# Autodesk Inventor assembly: PCB_board_box_reassemb
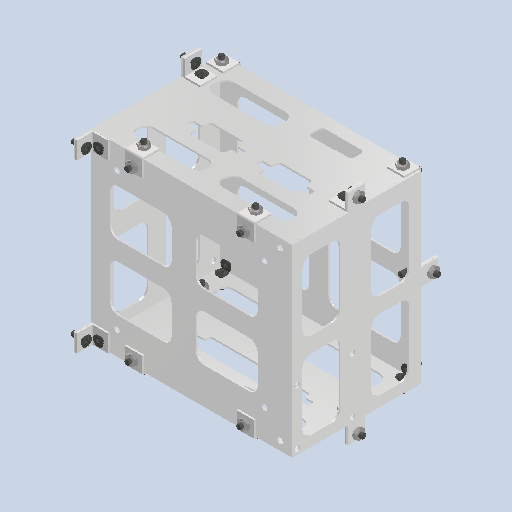
[picture p0: Inventor's stored thumbnail of the model, 512x512]
Saved by Autodesk Inventor 2023 (Build 270158000, 158)
## iProperties
Created: 2023-10-19
Part Number: PCB_board_box_reassemb
Document SubType Name: Assembly
Designer: 310611102
Author: 310611102
## Documents named in this file (10)
- C:\Users\310611102\Documents\Inventor\SSR\avionics_2023ver\electronics\shield box\shieldbox_ver2\PCB_board_box_reassemb.iam
- C:\Users\310611102\Documents\Inventor\SSR\avionics_2023ver\electronics\shield box\shieldbox_ver2\PCB_board_box_buttom.ipt
- C:\Users\310611102\Documents\Inventor\SSR\avionics_2023ver\electronics\shield box\shieldbox_ver2\PCB_board_box_front.ipt
- C:\Users\310611102\Documents\Inventor\SSR\avionics_2023ver\electronics\shield box\shieldbox_ver2\PCB_board_box_back.ipt
- C:\Users\310611102\Documents\Inventor\SSR\avionics_2023ver\electronics\shield box\shieldbox_ver2\PCB_board_box_right.ipt
- C:\Users\310611102\Documents\Inventor\SSR\avionics_2023ver\electronics\shield box\shieldbox_ver2\PCB_board_box_top.ipt
- C:\Users\310611102\Documents\Inventor\SSR\avionics_2023ver\electronics\shield box\shieldbox_ver2\PCB_board_box_left.ipt
- C:\Users\310611102\Documents\Inventor\SSR\avionics_2023ver\electronics\shield box\shieldbox_ver2\connector.ipt
- C:\Users\310611102\Documents\Inventor\SSR\avionics_2023ver\electronics\ISO 4032 - M3 - ISO.ipt
- C:\Users\310611102\Documents\Inventor\SSR\avionics_2023ver\electronics\ISO 10642 - M3 x  8.ipt
## Components (76 placed, 9 different names)
1. PCB_board_box_buttom:1 — Insert:16, Insert:18, Cylindrical:1, Cylindrical:3, Cylindrical:5, Cylindrical:9, Insert:53, Insert:55, Insert:57, Insert:59, Insert:85, Insert:87
2. PCB_board_box_front:1 — Insert:8, Insert:19, Cylindrical:4, Cylindrical:10, Cylindrical:13, Cylindrical:19, Insert:48, Insert:58, Insert:60, Insert:62, Insert:79, Insert:101
3. PCB_board_box_back:1 — Insert:27, Insert:41, Cylindrical:6, Cylindrical:11, Cylindrical:14, Cylindrical:16, Insert:50, Insert:51, Insert:54, Insert:56, Insert:83, Insert:100
4. PCB_board_box_right:1 — Insert:7, Insert:29, Insert:30, Insert:102, Insert:103, Insert:104
5. PCB_board_box_top:1 — Cylindrical:12, Insert:45, Cylindrical:15, Cylindrical:17, Cylindrical:18, Insert:46, Insert:49, Insert:52, Insert:61
6. PCB_board_box_left:1 — Insert:21, Insert:22, Insert:43, Insert:44
7. connector:1 — Cylindrical:3, Cylindrical:4, Insert:88, Insert:89
8. connector:3 — Insert:7, Insert:8, Insert:67, Insert:68
9. connector:4 — Insert:30, Insert:41, Insert:65, Insert:66
10. connector:5 — Cylindrical:5, Cylindrical:6, Insert:98, Insert:99
11. connector:6 — Cylindrical:1, Cylindrical:11, Insert:90, Insert:91
12. connector:7 — Insert:16, Insert:21, Insert:71, Insert:72
13. connector:8 — Insert:18, Insert:22, Insert:73, Insert:74
14. connector:9 — Insert:19, Insert:44, Insert:69, Insert:70
15. connector:12 — Insert:27, Insert:43, Insert:75, Insert:76
16. connector:13 — Insert:29, Insert:45, Insert:63, Insert:64
17. connector:14 — Cylindrical:16, Cylindrical:17, Insert:92, Insert:93
18. connector:15 — Cylindrical:14, Cylindrical:15, Insert:80, Insert:81
19. connector:16 — Cylindrical:12, Cylindrical:13, Insert:47, Insert:77
20. connector:18 — Cylindrical:9, Cylindrical:10, Insert:96, Insert:97
21. connector:19 — Cylindrical:18, Cylindrical:19, Insert:94, Insert:95
22. ISO 10642 M3x8:1 — Insert:46
23. ISO 10642 M3x8:2 — Insert:48
24. ISO 10642 M3x8:3 — Insert:49
25. ISO 10642 M3x8:4 — Insert:50
26. ISO 10642 M3x8:5 — Insert:51
27. ISO 10642 M3x8:6 — Insert:52
28. ISO 10642 M3x8:7 — Insert:53
29. ISO 10642 M3x8:8 — Insert:54
30. ISO 10642 M3x8:9 — Insert:55
31. ISO 10642 M3x8:10 — Insert:56
32. ISO 10642 M3x8:11 — Insert:57
33. ISO 10642 M3x8:12 — Insert:58
34. ISO 10642 M3x8:13 — Insert:59
35. ISO 10642 M3x8:14 — Insert:60
36. ISO 10642 M3x8:15 — Insert:61
37. ISO 10642 M3x8:16 — Insert:62
38. ISO 10642 M3x8:17 — Insert:63
39. ISO 10642 M3x8:18 — Insert:64
40. ISO 10642 M3x8:19 — Insert:65
41. ISO 10642 M3x8:20 — Insert:66
42. ISO 10642 M3x8:21 — Insert:67
43. ISO 10642 M3x8:22 — Insert:68
44. ISO 10642 M3x8:23 — Insert:69
45. ISO 10642 M3x8:24 — Insert:70
46. ISO 10642 M3x8:25 — Insert:71
47. ISO 10642 M3x8:26 — Insert:72
48. ISO 10642 M3x8:27 — Insert:73
49. ISO 10642 M3x8:28 — Insert:74
50. ISO 10642 M3x8:29 — Insert:75
51. ISO 10642 M3x8:30 — Insert:76
52. ISO 4032 M3:1 — Insert:47
53. ISO 4032 M3:2 — Insert:77
54. ISO 4032 M3:4 — Insert:79
55. ISO 4032 M3:5 — Insert:80
56. ISO 4032 M3:6 — Insert:81
57. ISO 4032 M3:8 — Insert:83
58. ISO 4032 M3:10 — Insert:85
59. ISO 4032 M3:12 — Insert:87
60. ISO 4032 M3:13 — Insert:88
61. ISO 4032 M3:14 — Insert:89
62. ISO 4032 M3:15 — Insert:90
63. ISO 4032 M3:16 — Insert:91
64. ISO 4032 M3:17 — Insert:92
65. ISO 4032 M3:18 — Insert:93
66. ISO 4032 M3:19 — Insert:94
67. ISO 4032 M3:20 — Insert:95
68. ISO 4032 M3:21 — Insert:96
69. ISO 4032 M3:22 — Insert:97
70. ISO 4032 M3:23 — Insert:98
71. ISO 4032 M3:24 — Insert:99
72. ISO 4032 M3:25 — Insert:100
73. ISO 4032 M3:26 — Insert:101
74. ISO 4032 M3:27 — Insert:102
75. ISO 4032 M3:28 — Insert:103
76. ISO 4032 M3:29 — Insert:104
## Relationships (85: Insert 69, CylindricalJoint 16)
- Insert:7: PCB_board_box_right:1 ↔ connector:3
- Insert:8: PCB_board_box_front:1 ↔ connector:3
- Insert:16: PCB_board_box_buttom:1 ↔ connector:7
- Insert:18: PCB_board_box_buttom:1 ↔ connector:8
- Insert:19: PCB_board_box_front:1 ↔ connector:9
- Insert:21: PCB_board_box_left:1 ↔ connector:7
- Insert:22: PCB_board_box_left:1 ↔ connector:8
- Insert:27: PCB_board_box_back:1 ↔ connector:12
- Insert:29: PCB_board_box_right:1 ↔ connector:13
- Insert:30: PCB_board_box_right:1 ↔ connector:4
- Insert:41: PCB_board_box_back:1 ↔ connector:4
- Cylindrical:1: PCB_board_box_buttom:1 ↔ connector:6
- Cylindrical:3: PCB_board_box_buttom:1 ↔ connector:1
- Cylindrical:4: PCB_board_box_front:1 ↔ connector:1
- Cylindrical:5: PCB_board_box_buttom:1 ↔ connector:5
- Cylindrical:6: PCB_board_box_back:1 ↔ connector:5
- Insert:43: PCB_board_box_left:1 ↔ connector:12
- Insert:44: PCB_board_box_left:1 ↔ connector:9
- Cylindrical:9: PCB_board_box_buttom:1 ↔ connector:18
- Cylindrical:10: PCB_board_box_front:1 ↔ connector:18
- Cylindrical:11: PCB_board_box_back:1 ↔ connector:6
- Cylindrical:12: PCB_board_box_top:1 ↔ connector:16
- Cylindrical:13: PCB_board_box_front:1 ↔ connector:16
- Insert:45: PCB_board_box_top:1 ↔ connector:13
- Cylindrical:14: PCB_board_box_back:1 ↔ connector:15
- Cylindrical:15: PCB_board_box_top:1 ↔ connector:15
- Cylindrical:16: PCB_board_box_back:1 ↔ connector:14
- Cylindrical:17: PCB_board_box_top:1 ↔ connector:14
- Cylindrical:18: PCB_board_box_top:1 ↔ connector:19
- Cylindrical:19: PCB_board_box_front:1 ↔ connector:19
- Insert:46: PCB_board_box_top:1 ↔ ISO 10642 M3x8:1
- Insert:47: connector:16 ↔ ISO 4032 M3:1
- Insert:48: PCB_board_box_front:1 ↔ ISO 10642 M3x8:2
- Insert:49: PCB_board_box_top:1 ↔ ISO 10642 M3x8:3
- Insert:50: PCB_board_box_back:1 ↔ ISO 10642 M3x8:4
- Insert:51: PCB_board_box_back:1 ↔ ISO 10642 M3x8:5
- Insert:52: PCB_board_box_top:1 ↔ ISO 10642 M3x8:6
- Insert:53: PCB_board_box_buttom:1 ↔ ISO 10642 M3x8:7
- Insert:54: PCB_board_box_back:1 ↔ ISO 10642 M3x8:8
- Insert:55: PCB_board_box_buttom:1 ↔ ISO 10642 M3x8:9
- Insert:56: PCB_board_box_back:1 ↔ ISO 10642 M3x8:10
- Insert:57: PCB_board_box_buttom:1 ↔ ISO 10642 M3x8:11
- Insert:58: PCB_board_box_front:1 ↔ ISO 10642 M3x8:12
- Insert:59: PCB_board_box_buttom:1 ↔ ISO 10642 M3x8:13
- Insert:60: PCB_board_box_front:1 ↔ ISO 10642 M3x8:14
- Insert:61: PCB_board_box_top:1 ↔ ISO 10642 M3x8:15
- Insert:62: PCB_board_box_front:1 ↔ ISO 10642 M3x8:16
- Insert:63: connector:13 ↔ ISO 10642 M3x8:17
- Insert:64: connector:13 ↔ ISO 10642 M3x8:18
- Insert:65: connector:4 ↔ ISO 10642 M3x8:19
- Insert:66: connector:4 ↔ ISO 10642 M3x8:20
- Insert:67: connector:3 ↔ ISO 10642 M3x8:21
- Insert:68: connector:3 ↔ ISO 10642 M3x8:22
- Insert:69: connector:9 ↔ ISO 10642 M3x8:23
- Insert:70: connector:9 ↔ ISO 10642 M3x8:24
- Insert:71: connector:7 ↔ ISO 10642 M3x8:25
- Insert:72: connector:7 ↔ ISO 10642 M3x8:26
- Insert:73: connector:8 ↔ ISO 10642 M3x8:27
- Insert:74: connector:8 ↔ ISO 10642 M3x8:28
- Insert:75: connector:12 ↔ ISO 10642 M3x8:29
- Insert:76: connector:12 ↔ ISO 10642 M3x8:30
- Insert:77: connector:16 ↔ ISO 4032 M3:2
- Insert:79: PCB_board_box_front:1 ↔ ISO 4032 M3:4
- Insert:80: connector:15 ↔ ISO 4032 M3:5
- Insert:81: connector:15 ↔ ISO 4032 M3:6
- Insert:83: PCB_board_box_back:1 ↔ ISO 4032 M3:8
- Insert:85: PCB_board_box_buttom:1 ↔ ISO 4032 M3:10
- Insert:87: PCB_board_box_buttom:1 ↔ ISO 4032 M3:12
- Insert:88: connector:1 ↔ ISO 4032 M3:13
- Insert:89: connector:1 ↔ ISO 4032 M3:14
- Insert:90: connector:6 ↔ ISO 4032 M3:15
- Insert:91: connector:6 ↔ ISO 4032 M3:16
- Insert:92: connector:14 ↔ ISO 4032 M3:17
- Insert:93: connector:14 ↔ ISO 4032 M3:18
- Insert:94: connector:19 ↔ ISO 4032 M3:19
- Insert:95: connector:19 ↔ ISO 4032 M3:20
- Insert:96: connector:18 ↔ ISO 4032 M3:21
- Insert:97: connector:18 ↔ ISO 4032 M3:22
- Insert:98: connector:5 ↔ ISO 4032 M3:23
- Insert:99: connector:5 ↔ ISO 4032 M3:24
- Insert:100: PCB_board_box_back:1 ↔ ISO 4032 M3:25
- Insert:101: PCB_board_box_front:1 ↔ ISO 4032 M3:26
- Insert:102: PCB_board_box_right:1 ↔ ISO 4032 M3:27
- Insert:103: PCB_board_box_right:1 ↔ ISO 4032 M3:28
- Insert:104: PCB_board_box_right:1 ↔ ISO 4032 M3:29
